# Autodesk Inventor assembly: Assey-N-N-body
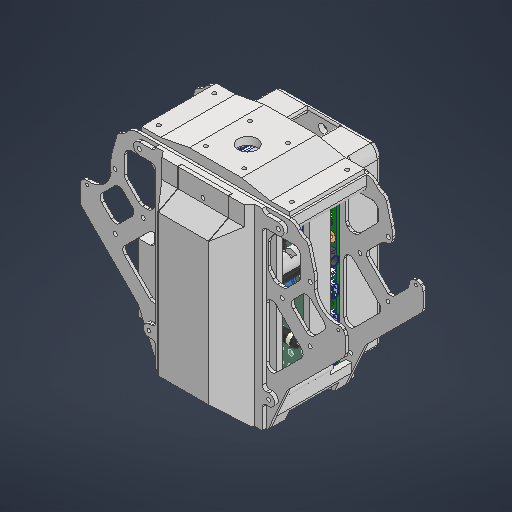
[picture p0: Inventor's stored thumbnail of the model, 512x512]
Saved by Autodesk Inventor 2026.1 (Build 301233020, 233B)
## iProperties
Created: 2026-03-17
Part Number: Assey-N-N-body
Document SubType Name: Assembly
Designer: kamada
Author: kamada
## Documents named in this file (10)
- D:\KiCad\KiProject\Nexus\Nexus-3dmodel\Assey-N-N-body.iam
- D:\KiCad\KiProject\Nexus\Nexus-3dmodel\NewBody-back.ipt
- D:\KiCad\KiProject\Nexus\Nexus-3dmodel\Nexus-pcb.iam
- D:\KiCad\KiProject\Nexus\Nexus-3dmodel\N-NBody.ipt
- D:\KiCad\KiProject\Nexus\Nexus-3dmodel\NewBody.ipt
- D:\KiCad\KiProject\Nexus\Nexus-3dmodel\NNFront.ipt
- D:\KiCad\KiProject\Nexus\Nexus-3dmodel\NNfront-huta.ipt
- D:\KiCad\KiProject\Nexus\Nexus-3dmodel\daiza.ipt
- D:\KiCad\KiProject\Nexus\Nexus-3dmodel\WMR-433-BK.ipt
- D:\KiCad\KiProject\Nexus\Nexus-3dmodel\NN-Ura.ipt
## Components (9 placed, 9 different names)
1. NewBody-back:1 — メイト:5, メイト:6, メイト:7, メイト:8, メイト:15, メイト:16, フラッシュ:3, フラッシュ:4, フラッシュ:5, メイト:29, フラッシュ:6, フラッシュ:7, フラッシュ:8
2. Nexus-pcb:1 [sub-assembly] — メイト:1, メイト:2, メイト:3, メイト:4, メイト:15, メイト:16
3. N-NBody:1 — フラッシュ:3, フラッシュ:4, フラッシュ:5, メイト:17, メイト:18, メイト:19, メイト:26, メイト:27, メイト:28
4. NewBody:1 — メイト:17, メイト:18, メイト:19, メイト:20, メイト:21, メイト:22
5. NNFront:1 — メイト:20, メイト:21, メイト:22, メイト:23, メイト:24, メイト:25
6. NNfront-huta:1 — メイト:23, メイト:24, メイト:25
7. daiza:1 — メイト:26, メイト:27, メイト:28
8. WMR-433-BK:1 — メイト:29, メイト:30, 角度:1
9. NN-Ura:1 — フラッシュ:6, フラッシュ:7, フラッシュ:8
## Relationships (36: Mate 27, Flush 6, Symmetry 2, Angle 1)
- メイト:1 [Mate]: Nexus-pcb:1
- メイト:2 [Mate]: Nexus-pcb:1
- メイト:3 [Mate]: Nexus-pcb:1
- メイト:4 [Mate]: Nexus-pcb:1
- 対称度:1 [Symmetry]
- メイト:5 [Mate]: NewBody-back:1
- メイト:6 [Mate]: NewBody-back:1
- メイト:7 [Mate]: NewBody-back:1
- メイト:8 [Mate]: NewBody-back:1
- 対称度:2 [Symmetry]
- メイト:9 [Mate]
- メイト:14 [Mate]
- メイト:15 [Mate] (3 mm): NewBody-back:1 ↔ Nexus-pcb:1
- メイト:16 [Mate] (1 mm): NewBody-back:1 ↔ Nexus-pcb:1
- フラッシュ:3 [Flush]: NewBody-back:1 ↔ N-NBody:1
- フラッシュ:4 [Flush]: NewBody-back:1 ↔ N-NBody:1
- フラッシュ:5 [Flush]: NewBody-back:1 ↔ N-NBody:1
- メイト:17 [Mate]: N-NBody:1 ↔ NewBody:1
- メイト:18 [Mate]: N-NBody:1 ↔ NewBody:1
- メイト:19 [Mate]: N-NBody:1 ↔ NewBody:1
- メイト:20 [Mate]: NewBody:1 ↔ NNFront:1
- メイト:21 [Mate]: NewBody:1 ↔ NNFront:1
- メイト:22 [Mate]: NewBody:1 ↔ NNFront:1
- メイト:23 [Mate]: NNFront:1 ↔ NNfront-huta:1
- メイト:24 [Mate]: NNFront:1 ↔ NNfront-huta:1
- メイト:25 [Mate]: NNFront:1 ↔ NNfront-huta:1
- メイト:26 [Mate]: N-NBody:1 ↔ daiza:1
- メイト:27 [Mate]: N-NBody:1 ↔ daiza:1
- メイト:28 [Mate]: N-NBody:1 ↔ daiza:1
- メイト:29 [Mate]: NewBody-back:1 ↔ WMR-433-BK:1
- メイト:30 [Mate]: WMR-433-BK:1
- 角度:1 [Angle] (0 deg): WMR-433-BK:1
- メイト:31 [Mate]
- フラッシュ:6 [Flush]: NewBody-back:1 ↔ NN-Ura:1
- フラッシュ:7 [Flush]: NewBody-back:1 ↔ NN-Ura:1
- フラッシュ:8 [Flush]: NewBody-back:1 ↔ NN-Ura:1
